# Autodesk Inventor assembly: AM14U3+Long+REV1-1
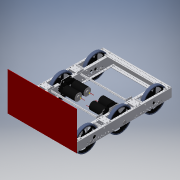
[picture p0: Inventor's stored thumbnail of the model, 180x180]
Saved by Autodesk Inventor 2016 (Build 200138000, 138)
## iProperties
Created: 2015-12-07
Part Number: AM14U3+Long+REV1-1
Description: STEP AP214
Document SubType Name: Assembly
Designer: Douglas
Sending System: SolidWorks 2014
Preprocessor: SwSTEP 2.0
Title: AM14U3 Long REV2.STEP
Revision Number: ANY
## Documents named in this file (3)
- D:\Douglas\Documents\Git\2016-Robot-CAD\Inventor\Chassis\AM14U3+Long+REV1-1.iam
- D:\Douglas\Documents\Git\2016-Robot-CAD\Inventor\Chassis\AM14U3 Long Half.iam
- D:\Douglas\Documents\Git\2016-Robot-CAD\Inventor\PARTS\TMP.ipt
## Components (3 placed, 3 different names)
1. AM14U3 Long Half_1 [sub-assembly] — Mate:1, Mate:2, Mate:3
2. AM14U3 Long Half_2 [sub-assembly] — Mate:1, Mate:2, Mate:3, Mate:4, Flush:1, Flush:2, Mate:5
3. TMP:1 — Mate:4, Flush:1, Flush:2
## Relationships (7: Mate 5, Flush 2)
- Mate:1: AM14U3 Long Half_1 ↔ AM14U3 Long Half_2
- Mate:2: AM14U3 Long Half_1 ↔ AM14U3 Long Half_2
- Mate:3: AM14U3 Long Half_1 ↔ AM14U3 Long Half_2
- Mate:4: AM14U3 Long Half_2 ↔ TMP:1
- Flush:1: AM14U3 Long Half_2 ↔ TMP:1
- Flush:2: AM14U3 Long Half_2 ↔ TMP:1
- Mate:5 (80.391 mm): AM14U3 Long Half_2
